# Autodesk Inventor assembly: Assembly2
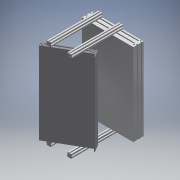
[picture p0: Inventor's stored thumbnail of the model, 180x180]
Saved by Autodesk Inventor 2016 (Build 200138000, 138)
## iProperties
Created: 2015-09-03
Part Number: Assembly2
Document SubType Name: Assembly
Designer: oscar
Author: oscar
## Documents named in this file (8)
- E:\documents\robocup-at-work\models\arena\elements\platform\shelf\inventor\shelf_assembly.iam
- E:\documents\robocup-at-work\models\arena\elements\platform\shelf\inventor\platform_800x500x99.ipt
- E:\documents\robocup-at-work\models\arena\elements\platform\shelf\inventor\B4040_500.ipt
- E:\documents\robocup-at-work\models\arena\elements\platform\shelf\inventor\bed_6mm.ipt
- E:\documents\robocup-at-work\models\arena\elements\platform\shelf\inventor\bed_wall.ipt
- E:\documents\robocup-at-work\models\arena\elements\platform\shelf\inventor\B4040_800.ipt
- E:\documents\robocup-at-work\models\arena\elements\platform\shelf\inventor\B4040_320.ipt
- E:\documents\robocup-at-work\models\arena\elements\platform\shelf\inventor\B4040_plastic_cover.ipt
## Components (15 placed, 7 different names)
1. platform_800x500x99:1 — Mate:3, Mate:4, Flush:2, Flush:3, Flush:5, Mate:7, Flush:8, Angle:1, Mate:18, Mate:24, Mate:25, Mate:26
2. B4040_500:1 — Mate:4, Flush:3, Mate:5, Flush:7, Flush:8, Mate:22, Flush:21, Flush:22
3. B4040_500:2 — Mate:3, Flush:2, Mate:5, Mate:21, Flush:19, Flush:20
4. B4040_500:3 — Flush:4, Flush:6, Mate:6, Mate:17, Mate:19, Flush:15, Flush:16, Mate:23
5. B4040_500:4 — Flush:4, Flush:5, Flush:6, Mate:6, Mate:7, Flush:7, Mate:20, Flush:17, Flush:18
6. bed_6mm:1 — Mate:8, Flush:9, Mate:9, Flush:10, Mate:10, Flush:12, Mate:13, Mate:15, Angle:1, Flush:14
7. bed_wall:1 — Mate:8, Flush:9, Mate:11, Flush:13, Mate:18, Mate:23
8. B4040_800:1 — Flush:12, Mate:13, Mate:14
9. B4040_800:2 — Mate:10, Mate:11, Flush:11, Mate:12, Mate:16, Flush:13
10. B4040_320:1 — Mate:9, Flush:10, Flush:11, Mate:12, Mate:14, Mate:17
11. B4040_320:2 — Mate:15, Mate:16, Flush:14
12. B4040_plastic_cover:1 — Mate:19, Flush:15, Flush:16
13. B4040_plastic_cover:2 — Mate:20, Flush:17, Flush:18
14. B4040_plastic_cover:3 — Mate:22, Flush:21, Flush:22
15. B4040_plastic_cover:4 — Mate:21, Flush:19, Flush:20
## Relationships (46: Mate 24, Flush 21, Angle 1)
- Mate:3: platform_800x500x99:1 ↔ B4040_500:2
- Mate:4: platform_800x500x99:1 ↔ B4040_500:1
- Flush:2: platform_800x500x99:1 ↔ B4040_500:2
- Flush:3: platform_800x500x99:1 ↔ B4040_500:1
- Mate:5 (160 mm): B4040_500:1 ↔ B4040_500:2
- Flush:4: B4040_500:3 ↔ B4040_500:4
- Flush:5: platform_800x500x99:1 ↔ B4040_500:4
- Flush:6: B4040_500:3 ↔ B4040_500:4
- Mate:6 (160 mm): B4040_500:3 ↔ B4040_500:4
- Mate:7: platform_800x500x99:1 ↔ B4040_500:4
- Flush:7: B4040_500:1 ↔ B4040_500:4
- Flush:8 (60 mm): platform_800x500x99:1 ↔ B4040_500:1
- Mate:8: bed_6mm:1 ↔ bed_wall:1
- Flush:9: bed_6mm:1 ↔ bed_wall:1
- Mate:9: bed_6mm:1 ↔ B4040_320:1
- Flush:10: bed_6mm:1 ↔ B4040_320:1
- Mate:10: bed_6mm:1 ↔ B4040_800:2
- Mate:11: bed_wall:1 ↔ B4040_800:2
- Flush:11: B4040_800:2 ↔ B4040_320:1
- Mate:12: B4040_800:2 ↔ B4040_320:1
- Flush:12: bed_6mm:1 ↔ B4040_800:1
- Mate:13: bed_6mm:1 ↔ B4040_800:1
- Mate:14: B4040_800:1 ↔ B4040_320:1
- Mate:15: bed_6mm:1 ↔ B4040_320:2
- Mate:16: B4040_800:2 ↔ B4040_320:2
- Mate:17: B4040_500:3 ↔ B4040_320:1
- Flush:13: bed_wall:1 ↔ B4040_800:2
- Angle:1 (150 deg): platform_800x500x99:1 ↔ bed_6mm:1
- Mate:18 (200 mm): platform_800x500x99:1 ↔ bed_wall:1
- Flush:14: bed_6mm:1 ↔ B4040_320:2
- Mate:19: B4040_500:3 ↔ B4040_plastic_cover:1
- Flush:15: B4040_500:3 ↔ B4040_plastic_cover:1
- Flush:16: B4040_500:3 ↔ B4040_plastic_cover:1
- Mate:20: B4040_500:4 ↔ B4040_plastic_cover:2
- Flush:17: B4040_500:4 ↔ B4040_plastic_cover:2
- Flush:18: B4040_500:4 ↔ B4040_plastic_cover:2
- Mate:21: B4040_500:2 ↔ B4040_plastic_cover:4
- Flush:19: B4040_500:2 ↔ B4040_plastic_cover:4
- Flush:20: B4040_500:2 ↔ B4040_plastic_cover:4
- Mate:22: B4040_500:1 ↔ B4040_plastic_cover:3
- Flush:21: B4040_500:1 ↔ B4040_plastic_cover:3
- Flush:22: B4040_500:1 ↔ B4040_plastic_cover:3
- Mate:23 (55 mm): B4040_500:3 ↔ bed_wall:1
- Mate:24: platform_800x500x99:1
- Mate:25: platform_800x500x99:1
- Mate:26: platform_800x500x99:1
